# Autodesk Inventor assembly: pegboard with legs
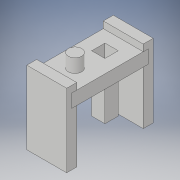
[picture p0: Inventor's stored thumbnail of the model, 180x180]
Saved by Autodesk Inventor 2018 (Build 220112000, 112)
## iProperties
Created: 2021-02-05
Part Number: pegboard with legs
Document SubType Name: Assembly
Designer: Bell539x
Author: Bell539x
## Documents named in this file (5)
- C:\Users\Bell539x\Downloads\pegboard with legs.iam
- C:\Users\Bell539x\Downloads\Pegboard.ipt
- C:\Users\Bell539x\Downloads\Cylinder.ipt
- C:\Users\Bell539x\Downloads\rectangular prism-01.ipt
- C:\Users\Bell539x\Downloads\leg.ipt
## Components (5 placed, 4 different names)
1. Pegboard:1 — Mate:1, Mate:2, Mate:3, Mate:4, Mate:5, Mate:6, Mate:7, Mate:8, Flush:1, Flush:2
2. Cylinder:1 — Mate:1, Mate:2
3. rectangular prism-01:1 — Mate:3, Mate:4
4. leg:1 — Mate:5, Mate:6, Flush:2
5. leg:2 — Mate:7, Mate:8, Flush:1
## Relationships (10: Mate 8, Flush 2)
- Mate:1: Pegboard:1 ↔ Cylinder:1
- Mate:2: Pegboard:1 ↔ Cylinder:1
- Mate:3: Pegboard:1 ↔ rectangular prism-01:1
- Mate:4: Pegboard:1 ↔ rectangular prism-01:1
- Mate:5: Pegboard:1 ↔ leg:1
- Mate:6: Pegboard:1 ↔ leg:1
- Mate:7: Pegboard:1 ↔ leg:2
- Mate:8: Pegboard:1 ↔ leg:2
- Flush:1: Pegboard:1 ↔ leg:2
- Flush:2: Pegboard:1 ↔ leg:1
